# Autodesk Inventor assembly: Vex Pro Ball Shifter 2 Stage  w US Digital Encoder
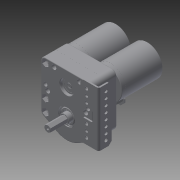
[picture p0: Inventor's stored thumbnail of the model, 180x180]
Saved by Autodesk Inventor 2014 (Build 180170000, 170)
## iProperties
Created: 2014-01-06
Part Number: Vex Pro Ball Shifter 2 Stage  w US Digital Encoder
Document SubType Name: Assembly
Designer: Andrew Toennies
Author: Andrew Toennies
Title: 217-2428 wUS Digital Encoder.20130115.STEP
Description: STEP AP203
Creation Date: 2013-01-14
Sending System: SolidWorks 2012
Preprocessor: SwSTEP 2.0
## Documents named in this file (32)
- C:\Users\Andrew Toennies\Documents\GitHub\2014buildCAD\Shooter\Vex Pro Ball Shifter 2 Stage  w US Digital Encoder.iam
- C:\Users\Andrew Toennies\Documents\GitHub\2014buildCAD\Imported Components\217-2428 wUS Digital Encoder.20130115\217-2733.ipt
- C:\Users\Andrew Toennies\Documents\GitHub\2014buildCAD\Imported Components\217-2428 wUS Digital Encoder.20130115\217-2731.ipt
- C:\Users\Andrew Toennies\Documents\GitHub\2014buildCAD\Imported Components\217-2428 wUS Digital Encoder.20130115\217-2789.ipt
- C:\Users\Andrew Toennies\Documents\GitHub\2014buildCAD\Imported Components\217-2428 wUS Digital Encoder.20130115\217-2778-001 Rev2_NCQ8A075-050M.iam
- C:\Users\Andrew Toennies\Documents\GitHub\2014buildCAD\Imported Components\217-2428 wUS Digital Encoder.20130115\217-2428-027 Rev1_97414A630.ipt
- C:\Users\Andrew Toennies\Documents\GitHub\2014buildCAD\Imported Components\217-2428 wUS Digital Encoder.20130115\217-2788_57155K375.ipt
- C:\Users\Andrew Toennies\Documents\GitHub\2014buildCAD\Imported Components\217-2428 wUS Digital Encoder.20130115\217-2428-012 Rev2.ipt
- C:\Users\Andrew Toennies\Documents\GitHub\2014buildCAD\Imported Components\217-2428 wUS Digital Encoder.20130115\217-2428-005 Rev1.ipt
- C:\Users\Andrew Toennies\Documents\GitHub\2014buildCAD\Imported Components\217-2428 wUS Digital Encoder.20130115\SCREW-832-0375.ipt
- C:\Users\Andrew Toennies\Documents\GitHub\2014buildCAD\Imported Components\217-2428 wUS Digital Encoder.20130115\SBS1_SBS-0632-0250.ipt
- C:\Users\Andrew Toennies\Documents\GitHub\2014buildCAD\Imported Components\217-2428 wUS Digital Encoder.20130115\217-2428-031 Rev1.iam
- C:\Users\Andrew Toennies\Documents\GitHub\2014buildCAD\Imported Components\217-2428 wUS Digital Encoder.20130115\217-2428-016 Rev2_Spur01.ipt
- C:\Users\Andrew Toennies\Documents\GitHub\2014buildCAD\Imported Components\217-2428 wUS Digital Encoder.20130115\217-2428-018 Rev2.ipt
- C:\Users\Andrew Toennies\Documents\GitHub\2014buildCAD\Imported Components\217-2428 wUS Digital Encoder.20130115\217-2428-009 Rev1.ipt
- C:\Users\Andrew Toennies\Documents\GitHub\2014buildCAD\Imported Components\217-2428 wUS Digital Encoder.20130115\SCREW-832-0250.ipt
- C:\Users\Andrew Toennies\Documents\GitHub\2014buildCAD\Imported Components\217-2428 wUS Digital Encoder.20130115\217-2428-024 Rev2.ipt
- C:\Users\Andrew Toennies\Documents\GitHub\2014buildCAD\Imported Components\217-2428 wUS Digital Encoder.20130115\SBS1_SBS1032-0500ZC.ipt
- C:\Users\Andrew Toennies\Documents\GitHub\2014buildCAD\Imported Components\217-2428 wUS Digital Encoder.20130115\217-2614-001_12t.ipt
- C:\Users\Andrew Toennies\Documents\GitHub\2014buildCAD\Imported Components\217-2428 wUS Digital Encoder.20130115\217-2761-001 rev1.ipt
- C:\Users\Andrew Toennies\Documents\GitHub\2014buildCAD\Imported Components\217-2428 wUS Digital Encoder.20130115\217-2428-001 Rev1.ipt
- C:\Users\Andrew Toennies\Documents\GitHub\2014buildCAD\Imported Components\217-2428 wUS Digital Encoder.20130115\217-2428-002 Rev2.ipt
- C:\Users\Andrew Toennies\Documents\GitHub\2014buildCAD\Imported Components\217-2428 wUS Digital Encoder.20130115\217-2703-001.ipt
- C:\Users\Andrew Toennies\Documents\GitHub\2014buildCAD\Imported Components\217-2428 wUS Digital Encoder.20130115\217-2707-001_40t.ipt
- C:\Users\Andrew Toennies\Documents\GitHub\2014buildCAD\Imported Components\217-2428 wUS Digital Encoder.20130115\Nylock Nut_NNY2520-ZC.ipt
- C:\Users\Andrew Toennies\Documents\GitHub\2014buildCAD\Imported Components\217-2428 wUS Digital Encoder.20130115\217-2428-004 Rev3.ipt
- C:\Users\Andrew Toennies\Documents\GitHub\2014buildCAD\Imported Components\217-2428 wUS Digital Encoder.20130115\217-2428-021 Rev1.ipt
- C:\Users\Andrew Toennies\Documents\GitHub\2014buildCAD\Imported Components\217-2428 wUS Digital Encoder.20130115\217-2428-029 Rev1.ipt
- C:\Users\Andrew Toennies\Documents\GitHub\2014buildCAD\Imported Components\217-2428 wUS Digital Encoder.20130115\217-2792-001 Rev1.iam
- C:\Users\Andrew Toennies\Documents\GitHub\2014buildCAD\Imported Components\217-2428 wUS Digital Encoder.20130115\E4P-X-250-X-D-D-D-X.ipt
- C:\Users\Andrew Toennies\Documents\GitHub\2014buildCAD\Imported Components\217-2428 wUS Digital Encoder.20130115\217-2428-200 Rev1.iam
- C:\Users\Andrew Toennies\Documents\GitHub\2014buildCAD\Shooter\minicim.ipt
## Components (49 placed, 48 different names)
1. 217-2733_1
2. 217-2733_2
3. 217-2731_3
4. 217-2789_4
5. 217-2778-001 Rev2_NCQ8A075-050M_5 [sub-assembly]
6. 217-2428-027 Rev1_97414A630_6
7. 217-2788_57155K375_7
8. 217-2428-012 Rev2_8
9. 217-2428-027 Rev1_97414A630_9
10. 217-2428-005 Rev1_10
11. 217-2428-005 Rev1_11
12. SCREW-832-0375_12
13. SCREW-832-0375_13
14. SCREW-832-0375_14
15. SCREW-832-0375_15
16. SBS1_SBS-0632-0250_16
17. SBS1_SBS-0632-0250_17
18. 217-2428-031 Rev1_18 [sub-assembly]
19. 217-2428-016 Rev2_Spur01_19
20. 217-2428-018 Rev2_20
21. 217-2428-009 Rev1_21
22. 217-2428-009 Rev1_22
23. SCREW-832-0250_23
24. SCREW-832-0375_24
25. SCREW-832-0375_25
26. SCREW-832-0250_26
27. 217-2428-024 Rev2_27
28. SBS1_SBS1032-0500ZC_28
29. SBS1_SBS1032-0500ZC_29 — Mate:3
30. 217-2614-001_12t_30 — Mate:1
31. 217-2761-001 rev1_31
32. SBS1_SBS1032-0500ZC_32
33. SBS1_SBS1032-0500ZC_33 — Mate:4
34. 217-2761-001 rev1_34
35. 217-2614-001_12t_35 — Mate:2
36. 217-2428-001 Rev1_36 — Mate:5
37. 217-2428-002 Rev2_37
38. 217-2703-001_38
39. 217-2707-001_40t_39
40. Nylock Nut_NNY2520-ZC_40
41. Nylock Nut_NNY2520-ZC_41
42. 217-2428-004 Rev3_42
43. 217-2428-021 Rev1_43
44. 217-2428-029 Rev1_44
45. 217-2792-001 Rev1_45 [sub-assembly]
46. E4P-X-250-X-D-D-D-X_48
47. 217-2428-200 Rev1_49 [sub-assembly]
48. minicim:1 — Mate:1, Flush:1, Mate:3
49. minicim:2 — Mate:2, Flush:1, Mate:4, Mate:5
## Relationships (6: Mate 5, Flush 1)
- Mate:1: 217-2614-001_12t_30 ↔ minicim:1
- Mate:2: 217-2614-001_12t_35 ↔ minicim:2
- Flush:1: minicim:1 ↔ minicim:2
- Mate:3: SBS1_SBS1032-0500ZC_29 ↔ minicim:1
- Mate:4: SBS1_SBS1032-0500ZC_33 ↔ minicim:2
- Mate:5: 217-2428-001 Rev1_36 ↔ minicim:2
